# Autodesk Inventor assembly: nc_nhk12
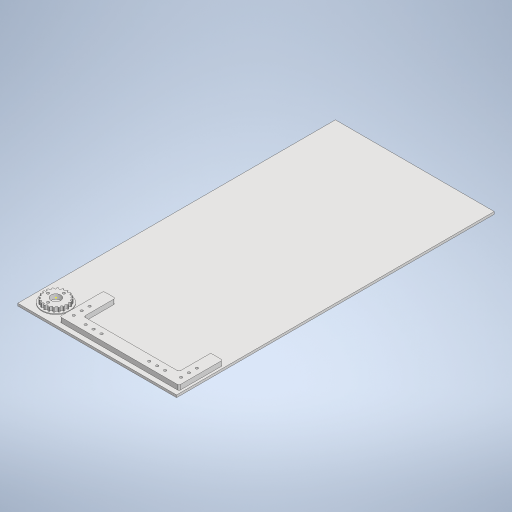
[picture p0: Inventor's stored thumbnail of the model, 512x512]
Saved by Autodesk Inventor 2023 (Build 270158000, 158)
## iProperties
Created: 2022-04-23
Part Number: nc_nhk12
Document SubType Name: Assembly
Designer: yuta
Author: yuta
## Documents named in this file (4)
- C:\Users\yuta\Documents\NHK\nc_nhk12.iam
- C:\Users\yuta\Documents\NHK\NC.port.ipt
- C:\Users\yuta\Documents\NHK\射出_プーリ_歯数20.ipt
- C:\Users\yuta\Documents\NHK\射出_受け身.ipt
## Components (3 placed, 3 different names)
1. NC.port:1 — メイト:1, メイト:2, メイト:3, フラッシュ:1, フラッシュ:2, メイト:4
2. 射出_プーリ_歯数20:1 — メイト:1, メイト:2, メイト:3
3. 射出_受け身:1 — フラッシュ:1, フラッシュ:2, メイト:4
## Relationships (6: Mate 4, Flush 2)
- メイト:1 [Mate]: NC.port:1 ↔ 射出_プーリ_歯数20:1
- メイト:2 [Mate] (-24 mm): NC.port:1 ↔ 射出_プーリ_歯数20:1
- メイト:3 [Mate] (-24 mm): NC.port:1 ↔ 射出_プーリ_歯数20:1
- フラッシュ:1 [Flush] (3 mm): NC.port:1 ↔ 射出_受け身:1
- フラッシュ:2 [Flush] (6 mm): NC.port:1 ↔ 射出_受け身:1
- メイト:4 [Mate]: NC.port:1 ↔ 射出_受け身:1
